# Autodesk Inventor assembly: Foot
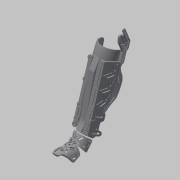
[picture p0: Inventor's stored thumbnail of the model, 180x180]
Saved by Autodesk Inventor 2015 SP1 (Build 190203100, 203)
## iProperties
Created: 2014-12-25
Part Number: Foot
Document SubType Name: Assembly
Designer: Val
Author: Val
## Documents named in this file (8)
- C:\Users\Val\Desktop\ExoGit\elysium-max-exoskeleton\src\assemblies\LegLeft.iam
- C:\Users\Val\Desktop\ExoGit\elysium-max-exoskeleton\src\FootShockPlate.ipt
- C:\Users\Val\Desktop\ExoGit\elysium-max-exoskeleton\src\FootUpperShockPlate.ipt
- C:\Users\Val\Desktop\ExoGit\elysium-max-exoskeleton\src\ShinConnectorLeft.ipt
- C:\Users\Val\Desktop\ExoGit\elysium-max-exoskeleton\src\ShinShockPlateLeft.ipt
- C:\Users\Val\Desktop\ExoGit\elysium-max-exoskeleton\src\ShinLeft.ipt
- C:\Users\Val\Desktop\ExoGit\elysium-max-exoskeleton\src\ShinLockLeft.ipt
- C:\Users\Val\Desktop\ExoGit\elysium-max-exoskeleton\src\ShinExtender.ipt
## Components (7 placed, 7 different names)
1. FootShockPlate:1
2. FootUpperShockPlate:1
3. ShinConnectorLeft:1 — Mate:7, Mate:8, Mate:9, Mate:10, Mate:11, Mate:12
4. ShinShockPlateLeft:1 — Mate:1, Mate:2, Mate:3
5. ShinLeft:1 — Mate:1, Mate:2, Mate:3, Mate:4, Mate:5, Mate:6, Mate:10, Mate:11, Mate:12
6. ShinLockLeft:1 — Mate:4, Mate:5, Mate:6
7. ShinExtender:2 — Mate:7, Mate:8, Mate:9
## Relationships (12: Mate 12)
- Mate:1: ShinShockPlateLeft:1 ↔ ShinLeft:1
- Mate:2: ShinShockPlateLeft:1 ↔ ShinLeft:1
- Mate:3: ShinShockPlateLeft:1 ↔ ShinLeft:1
- Mate:4: ShinLeft:1 ↔ ShinLockLeft:1
- Mate:5: ShinLeft:1 ↔ ShinLockLeft:1
- Mate:6: ShinLeft:1 ↔ ShinLockLeft:1
- Mate:7: ShinConnectorLeft:1 ↔ ShinExtender:2
- Mate:8: ShinConnectorLeft:1 ↔ ShinExtender:2
- Mate:9: ShinConnectorLeft:1 ↔ ShinExtender:2
- Mate:10: ShinConnectorLeft:1 ↔ ShinLeft:1
- Mate:11: ShinConnectorLeft:1 ↔ ShinLeft:1
- Mate:12: ShinConnectorLeft:1 ↔ ShinLeft:1
